# Autodesk Inventor assembly: Сборка1
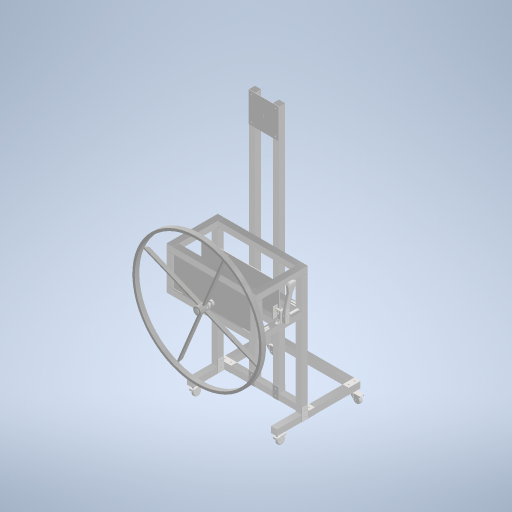
[picture p0: Inventor's stored thumbnail of the model, 512x512]
Saved by Autodesk Inventor 2023 (Build 270158000, 158)
## iProperties
Created: 2022-04-27
Part Number: Сборка1
Document SubType Name: Assembly
Designer: User
Author: User
## Documents named in this file (11)
- D:\Стойка\VR-simulator-3D-models\Стойка.iam
- D:\Стойка\VR-simulator-3D-models\Новый каркас.ipt
- D:\Стойка\VR-simulator-3D-models\Колесо.ipt
- D:\Стойка\VR-simulator-3D-models\Шпилька для ролика.ipt
- D:\Стойка\VR-simulator-3D-models\Соединитель 40х80.ipt
- D:\Стойка\VR-simulator-3D-models\Внутренний соединитель.ipt
- D:\Стойка\VR-simulator-3D-models\Угол 40х40.ipt
- D:\Стойка\VR-simulator-3D-models\Механизм ручки\Сборка ручка.iam
- D:\Стойка\VR-simulator-3D-models\Механизм ручки\угол (1).ipt
- D:\Стойка\VR-simulator-3D-models\Механизм\Сборка штурвал.iam
- D:\Стойка\VR-simulator-3D-models\Пластина.ipt
## Components (55 placed, 10 different names)
1. Новый каркас:1 — Совмещение:1, Заподлицо:1, Совмещение:2, Заподлицо:2, Совмещение:4, Заподлицо:5, Совмещение:5, Заподлицо:6, Совмещение:6, Совмещение:7, Заподлицо:7, Заподлицо:8, Заподлицо:9, Заподлицо:10, Совмещение:8, Совмещение:9, Заподлицо:11, Заподлицо:12, Заподлицо:13, Заподлицо:14, Заподлицо:15, Заподлицо:16, Заподлицо:17, Совмещение:10, Совмещение:11, Совмещение:12, Совмещение:13, Заподлицо:18, Заподлицо:19, Заподлицо:20, Заподлицо:21, Совмещение:14, Заподлицо:22, Совмещение:15, Заподлицо:23, Заподлицо:24, Заподлицо:25, Заподлицо:26, Заподлицо:27, Заподлицо:28, Заподлицо:29, Заподлицо:30, Совмещение:16, Заподлицо:31, Заподлицо:32, Заподлицо:33, Совмещение:17, Совмещение:18, Совмещение:19, Заподлицо:35, Заподлицо:36, Совмещение:21, Совмещение:22, Заподлицо:37, Совмещение:23, Совмещение:24, Совмещение:25, Совмещение:26, Совмещение:27, Совмещение:28, Совмещение:29, Совмещение:33, Совмещение:34, Совмещение:36, Совмещение:37, Совмещение:38, Совмещение:39, Совмещение:40, Заподлицо:46, Заподлицо:47, Заподлицо:48, Заподлицо:49, Заподлицо:50, Совмещение:46, Заподлицо:51, Совмещение:47, Заподлицо:52, Совмещение:48, Совмещение:49, Заподлицо:53, Заподлицо:54, Совмещение:50, Заподлицо:55, Заподлицо:56, Совмещение:51, Совмещение:52, Совмещение:53, Совмещение:56, Совмещение:57, Совмещение:62, Совмещение:63, Совмещение:64, Совмещение:65, Совмещение:66, Заподлицо:57, Заподлицо:58
2. Колесо:1 — С поворотом:2, С поворотом:10
3. Колесо:2 — С поворотом:6, С поворотом:8
4. Колесо:3 — С поворотом:4, С поворотом:9
5. Колесо:4 — С поворотом:3, С поворотом:7
6. Шпилька для ролика:1 — С поворотом:2, С поворотом:10
7. Шпилька для ролика:2 — С поворотом:3, С поворотом:7
8. Шпилька для ролика:3 — С поворотом:6, С поворотом:8
9. Шпилька для ролика:4 — С поворотом:4, С поворотом:9
10. Соединитель 40х80:1 — Совмещение:1, Заподлицо:1, Заподлицо:15
11. Соединитель 40х80:2 — Совмещение:2, Заподлицо:2
12. Соединитель 40х80:3 — Совмещение:6, Заподлицо:9, Заподлицо:10
13. Соединитель 40х80:4 — Совмещение:8, Заподлицо:11, Заподлицо:14
14. Соединитель 40х80:5 — Совмещение:5, Заподлицо:6, Заподлицо:17
15. Соединитель 40х80:6 — Совмещение:4, Заподлицо:5, Заподлицо:16
16. Соединитель 40х80:8 — Совмещение:7, Заподлицо:7, Заподлицо:8
17. Соединитель 40х80:10 — Совмещение:9, Заподлицо:12, Заподлицо:13
18. Соединитель 40х80:11 — Совмещение:10, Заподлицо:25, Заподлицо:26
19. Соединитель 40х80:12 — Совмещение:13, Заподлицо:18, Заподлицо:19
20. Соединитель 40х80:13 — Совмещение:14, Заподлицо:22, Заподлицо:29
21. Соединитель 40х80:14 — Совмещение:15, Заподлицо:23, Заподлицо:24
22. Соединитель 40х80:15 — Совмещение:11, Заподлицо:27, Заподлицо:28
23. Соединитель 40х80:16 — Совмещение:12, Заподлицо:20, Заподлицо:21
24. Внутренний соединитель:2 — Заподлицо:33, Совмещение:17
25. Внутренний соединитель:3 — Заподлицо:30, Совмещение:16
26. Внутренний соединитель:4 — Совмещение:24, Заподлицо:49
27. Внутренний соединитель:5 — Заподлицо:35, Совмещение:21
28. Внутренний соединитель:7 — Совмещение:28
29. Внутренний соединитель:8 — Совмещение:29, Заподлицо:48
30. Внутренний соединитель:9 — Совмещение:26
31. Внутренний соединитель:10 — Заподлицо:31, Совмещение:18
32. Внутренний соединитель:11 — Заподлицо:32, Совмещение:19
33. Внутренний соединитель:12 — Заподлицо:37, Совмещение:23
34. Внутренний соединитель:13 — Совмещение:27
35. Внутренний соединитель:14 — Совмещение:25
36. Внутренний соединитель:15 — Заподлицо:36, Совмещение:22
37. Угол 40х40:1 — Совмещение:36, Совмещение:37
38. Угол 40х40:2 — Совмещение:38, Совмещение:39
39. Угол 40х40:3 — Совмещение:33
40. Угол 40х40:4 — Совмещение:34
41. Сборка ручка:1 [sub-assembly] — Совмещение:40, Заподлицо:46, Совмещение:44, Заподлицо:47, Совмещение:54, Совмещение:55
42. угол (1):1 — Совмещение:44, Совмещение:51
43. Внутренний соединитель:17 — Заподлицо:51, Совмещение:47
44. Внутренний соединитель:18 — Заподлицо:50, Совмещение:46
45. Внутренний соединитель:19 — Заподлицо:52, Совмещение:48
46. Соединитель 40х80:17 — Совмещение:49, Заподлицо:53, Заподлицо:54
47. Соединитель 40х80:18 — Совмещение:50, Заподлицо:55, Заподлицо:56
48. угол (1):2 — Совмещение:52, Совмещение:54
49. угол (1):3 — Совмещение:53, Совмещение:55
50. Сборка штурвал:1 [sub-assembly] — Совмещение:56, Совмещение:57, Совмещение:58, Совмещение:59, Совмещение:60, Совмещение:61
51. угол (1):4 — Совмещение:58, Совмещение:65
52. угол (1):5 — Совмещение:59, Совмещение:64
53. угол (1):6 — Совмещение:61, Совмещение:62
54. угол (1):7 — Совмещение:60, Совмещение:63
55. Пластина:1 — Совмещение:66, Заподлицо:57, Заподлицо:58
## Relationships (111: Mate 56, Flush 47, RevoluteJoint 8)
- С поворотом:2 [RevoluteJoint]: Колесо:1 ↔ Шпилька для ролика:1
- С поворотом:3 [RevoluteJoint]: Колесо:4 ↔ Шпилька для ролика:2
- С поворотом:4 [RevoluteJoint]: Колесо:3 ↔ Шпилька для ролика:4
- С поворотом:6 [RevoluteJoint]: Колесо:2 ↔ Шпилька для ролика:3
- С поворотом:7 [RevoluteJoint]: Колесо:4 ↔ Шпилька для ролика:2
- С поворотом:8 [RevoluteJoint]: Колесо:2 ↔ Шпилька для ролика:3
- С поворотом:9 [RevoluteJoint]: Колесо:3 ↔ Шпилька для ролика:4
- С поворотом:10 [RevoluteJoint]: Колесо:1 ↔ Шпилька для ролика:1
- Совмещение:1 [Mate]: Новый каркас:1 ↔ Соединитель 40х80:1
- Заподлицо:1 [Flush]: Новый каркас:1 ↔ Соединитель 40х80:1
- Совмещение:2 [Mate]: Новый каркас:1 ↔ Соединитель 40х80:2
- Заподлицо:2 [Flush]: Новый каркас:1 ↔ Соединитель 40х80:2
- Совмещение:4 [Mate]: Новый каркас:1 ↔ Соединитель 40х80:6
- Заподлицо:5 [Flush]: Новый каркас:1 ↔ Соединитель 40х80:6
- Совмещение:5 [Mate]: Новый каркас:1 ↔ Соединитель 40х80:5
- Заподлицо:6 [Flush]: Новый каркас:1 ↔ Соединитель 40х80:5
- Совмещение:6 [Mate]: Новый каркас:1 ↔ Соединитель 40х80:3
- Совмещение:7 [Mate]: Новый каркас:1 ↔ Соединитель 40х80:8
- Заподлицо:7 [Flush]: Новый каркас:1 ↔ Соединитель 40х80:8
- Заподлицо:8 [Flush]: Новый каркас:1 ↔ Соединитель 40х80:8
- Заподлицо:9 [Flush]: Новый каркас:1 ↔ Соединитель 40х80:3
- Заподлицо:10 [Flush]: Новый каркас:1 ↔ Соединитель 40х80:3
- Совмещение:8 [Mate]: Новый каркас:1 ↔ Соединитель 40х80:4
- Совмещение:9 [Mate]: Новый каркас:1 ↔ Соединитель 40х80:10
- Заподлицо:11 [Flush]: Новый каркас:1 ↔ Соединитель 40х80:4
- Заподлицо:12 [Flush]: Новый каркас:1 ↔ Соединитель 40х80:10
- Заподлицо:13 [Flush]: Новый каркас:1 ↔ Соединитель 40х80:10
- Заподлицо:14 [Flush]: Новый каркас:1 ↔ Соединитель 40х80:4
- Заподлицо:15 [Flush]: Новый каркас:1 ↔ Соединитель 40х80:1
- Заподлицо:16 [Flush]: Новый каркас:1 ↔ Соединитель 40х80:6
- Заподлицо:17 [Flush]: Новый каркас:1 ↔ Соединитель 40х80:5
- Совмещение:10 [Mate]: Новый каркас:1 ↔ Соединитель 40х80:11
- Совмещение:11 [Mate]: Новый каркас:1 ↔ Соединитель 40х80:15
- Совмещение:12 [Mate]: Новый каркас:1 ↔ Соединитель 40х80:16
- Совмещение:13 [Mate]: Новый каркас:1 ↔ Соединитель 40х80:12
- Заподлицо:18 [Flush]: Новый каркас:1 ↔ Соединитель 40х80:12
- Заподлицо:19 [Flush]: Новый каркас:1 ↔ Соединитель 40х80:12
- Заподлицо:20 [Flush]: Новый каркас:1 ↔ Соединитель 40х80:16
- Заподлицо:21 [Flush]: Новый каркас:1 ↔ Соединитель 40х80:16
- Совмещение:14 [Mate]: Новый каркас:1 ↔ Соединитель 40х80:13
- Заподлицо:22 [Flush]: Новый каркас:1 ↔ Соединитель 40х80:13
- Совмещение:15 [Mate]: Новый каркас:1 ↔ Соединитель 40х80:14
- Заподлицо:23 [Flush]: Новый каркас:1 ↔ Соединитель 40х80:14
- Заподлицо:24 [Flush]: Новый каркас:1 ↔ Соединитель 40х80:14
- Заподлицо:25 [Flush]: Новый каркас:1 ↔ Соединитель 40х80:11
- Заподлицо:26 [Flush]: Новый каркас:1 ↔ Соединитель 40х80:11
- Заподлицо:27 [Flush]: Новый каркас:1 ↔ Соединитель 40х80:15
- Заподлицо:28 [Flush]: Новый каркас:1 ↔ Соединитель 40х80:15
- Заподлицо:29 [Flush]: Новый каркас:1 ↔ Соединитель 40х80:13
- Заподлицо:30 [Flush]: Новый каркас:1 ↔ Внутренний соединитель:3
- Совмещение:16 [Mate]: Новый каркас:1 ↔ Внутренний соединитель:3
- Заподлицо:31 [Flush]: Новый каркас:1 ↔ Внутренний соединитель:10
- Заподлицо:32 [Flush]: Новый каркас:1 ↔ Внутренний соединитель:11
- Заподлицо:33 [Flush]: Новый каркас:1 ↔ Внутренний соединитель:2
- Совмещение:17 [Mate]: Новый каркас:1 ↔ Внутренний соединитель:2
- Совмещение:18 [Mate]: Новый каркас:1 ↔ Внутренний соединитель:10
- Совмещение:19 [Mate]: Новый каркас:1 ↔ Внутренний соединитель:11
- Заподлицо:35 [Flush]: Новый каркас:1 ↔ Внутренний соединитель:5
- Заподлицо:36 [Flush]: Новый каркас:1 ↔ Внутренний соединитель:15
- Совмещение:21 [Mate]: Новый каркас:1 ↔ Внутренний соединитель:5
- Совмещение:22 [Mate]: Новый каркас:1 ↔ Внутренний соединитель:15
- Заподлицо:37 [Flush]: Новый каркас:1 ↔ Внутренний соединитель:12
- Совмещение:23 [Mate]: Новый каркас:1 ↔ Внутренний соединитель:12
- Совмещение:24 [Mate]: Новый каркас:1 ↔ Внутренний соединитель:4
- Совмещение:25 [Mate]: Новый каркас:1 ↔ Внутренний соединитель:14
- Совмещение:26 [Mate]: Новый каркас:1 ↔ Внутренний соединитель:9
- Совмещение:27 [Mate]: Новый каркас:1 ↔ Внутренний соединитель:13
- Совмещение:28 [Mate]: Новый каркас:1 ↔ Внутренний соединитель:7
- Совмещение:29 [Mate]: Новый каркас:1 ↔ Внутренний соединитель:8
- Совмещение:33 [Mate]: Новый каркас:1 ↔ Угол 40х40:3
- Совмещение:34 [Mate]: Новый каркас:1 ↔ Угол 40х40:4
- Совмещение:36 [Mate]: Новый каркас:1 ↔ Угол 40х40:1
- Совмещение:37 [Mate]: Новый каркас:1 ↔ Угол 40х40:1
- Совмещение:38 [Mate]: Новый каркас:1 ↔ Угол 40х40:2
- Совмещение:39 [Mate]: Новый каркас:1 ↔ Угол 40х40:2
- Совмещение:40 [Mate]: Новый каркас:1 ↔ Сборка ручка:1
- Заподлицо:46 [Flush]: Новый каркас:1 ↔ Сборка ручка:1
- Совмещение:44 [Mate]: Сборка ручка:1 ↔ угол (1):1
- Заподлицо:47 [Flush]: Новый каркас:1 ↔ Сборка ручка:1
- Заподлицо:48 [Flush]: Новый каркас:1 ↔ Внутренний соединитель:8
- Заподлицо:49 [Flush]: Новый каркас:1 ↔ Внутренний соединитель:4
- Заподлицо:50 [Flush]: Новый каркас:1 ↔ Внутренний соединитель:18
- Совмещение:46 [Mate]: Новый каркас:1 ↔ Внутренний соединитель:18
- Заподлицо:51 [Flush]: Новый каркас:1 ↔ Внутренний соединитель:17
- Совмещение:47 [Mate]: Новый каркас:1 ↔ Внутренний соединитель:17
- Заподлицо:52 [Flush]: Новый каркас:1 ↔ Внутренний соединитель:19
- Совмещение:48 [Mate]: Новый каркас:1 ↔ Внутренний соединитель:19
- Совмещение:49 [Mate]: Новый каркас:1 ↔ Соединитель 40х80:17
- Заподлицо:53 [Flush]: Новый каркас:1 ↔ Соединитель 40х80:17
- Заподлицо:54 [Flush]: Новый каркас:1 ↔ Соединитель 40х80:17
- Совмещение:50 [Mate]: Новый каркас:1 ↔ Соединитель 40х80:18
- Заподлицо:55 [Flush]: Новый каркас:1 ↔ Соединитель 40х80:18
- Заподлицо:56 [Flush]: Новый каркас:1 ↔ Соединитель 40х80:18
- Совмещение:51 [Mate]: Новый каркас:1 ↔ угол (1):1
- Совмещение:52 [Mate]: Новый каркас:1 ↔ угол (1):2
- Совмещение:53 [Mate]: Новый каркас:1 ↔ угол (1):3
- Совмещение:54 [Mate]: Сборка ручка:1 ↔ угол (1):2
- Совмещение:55 [Mate]: Сборка ручка:1 ↔ угол (1):3
- Совмещение:56 [Mate]: Новый каркас:1 ↔ Сборка штурвал:1
- Совмещение:57 [Mate]: Новый каркас:1 ↔ Сборка штурвал:1
- Совмещение:58 [Mate]: Сборка штурвал:1 ↔ угол (1):4
- Совмещение:59 [Mate]: Сборка штурвал:1 ↔ угол (1):5
- Совмещение:60 [Mate]: Сборка штурвал:1 ↔ угол (1):7
- Совмещение:61 [Mate]: Сборка штурвал:1 ↔ угол (1):6
- Совмещение:62 [Mate]: Новый каркас:1 ↔ угол (1):6
- Совмещение:63 [Mate]: Новый каркас:1 ↔ угол (1):7
- Совмещение:64 [Mate]: Новый каркас:1 ↔ угол (1):5
- Совмещение:65 [Mate]: Новый каркас:1 ↔ угол (1):4
- Совмещение:66 [Mate]: Новый каркас:1 ↔ Пластина:1
- Заподлицо:57 [Flush]: Новый каркас:1 ↔ Пластина:1
- Заподлицо:58 [Flush]: Новый каркас:1 ↔ Пластина:1
